# Autodesk Inventor assembly: Galileo Plate
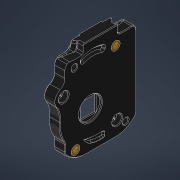
[picture p0: Inventor's stored thumbnail of the model, 180x180]
Saved by Autodesk Inventor 2022.2 (Build 262287010, 287A)
## iProperties
Created: 2022-03-15
Part Number: Galileo Plate
Document SubType Name: Assembly
Designer: sleib
Author: sleib
## Documents named in this file (3)
- C:\Users\sleib\Projekte\Voron-2\CAD\Inventor\Galileo Clockwork\Galileo Plate.iam
- C:\Users\sleib\Projekte\Voron-2\CAD\Inventor\Galileo Clockwork\Rear Plate.ipt
- C:\Users\sleib\Projekte\Voron-2\CAD\Inventor\M3 Threaded Insert.ipt
## Components (3 placed, 2 different names)
1. Rear Plate:1 — Passend:1, Passend:2, Fluchtend:1, Fluchtend:2
2. M3 Threaded Insert:1 — Passend:1, Fluchtend:2
3. M3 Threaded Insert:2 — Passend:2, Fluchtend:1
## Relationships (4: Mate 2, Flush 2)
- Passend:1 [Mate]: Rear Plate:1 ↔ M3 Threaded Insert:1
- Passend:2 [Mate]: Rear Plate:1 ↔ M3 Threaded Insert:2
- Fluchtend:1 [Flush]: Rear Plate:1 ↔ M3 Threaded Insert:2
- Fluchtend:2 [Flush]: Rear Plate:1 ↔ M3 Threaded Insert:1
